# Autodesk Inventor assembly: protecaoAcrilico
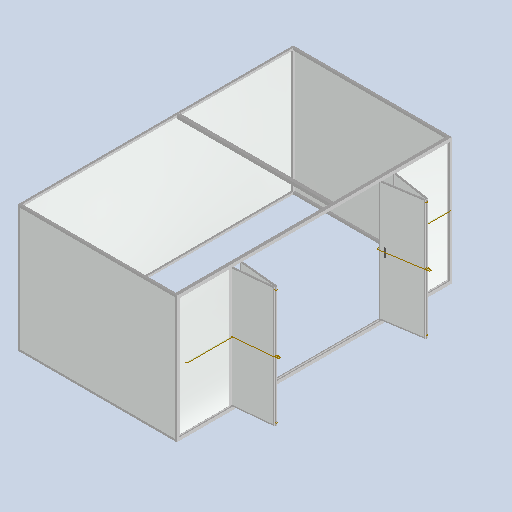
[picture p0: Inventor's stored thumbnail of the model, 512x512]
Saved by Autodesk Inventor 2023 (Build 270158000, 158)
## iProperties
Created: 2022-08-29
Part Number: protecaoAcrilico
Document SubType Name: Assembly
Designer: cvss2
Author: cvss2
## Documents named in this file (14)
- C:\Users\cvss2.CINSOFTEX\Documents\Residencia Softex 2021-2022\modelos 3D\Denso VS050\mesa2Denso\proteçao2Densos\protecaoAcrilico2Densos.iam
- C:\Users\cvss2.CINSOFTEX\Documents\Residencia Softex 2021-2022\modelos 3D\Denso VS050\mesa2Denso\proteçao2Densos\estrutura.ipt
- C:\Users\cvss2.CINSOFTEX\Documents\Residencia Softex 2021-2022\modelos 3D\Denso VS050\mesa2Denso\proteçao2Densos\acrilicoFixo.ipt
- C:\Users\cvss2.CINSOFTEX\Documents\Residencia Softex 2021-2022\modelos 3D\Denso VS050\mesa2Denso\proteçao2Densos\acrilicoFixo2.ipt
- C:\Users\cvss2.CINSOFTEX\Documents\Residencia Softex 2021-2022\modelos 3D\Denso VS050\mesa2Denso\proteçao2Densos\guiaPorta.ipt
- C:\Users\cvss2.CINSOFTEX\Documents\Residencia Softex 2021-2022\modelos 3D\Denso VS050\mesa2Denso\madeiraMesa.ipt
- C:\Users\cvss2.CINSOFTEX\Documents\Residencia Softex 2021-2022\modelos 3D\Denso VS050\mesa2Denso\proteçao2Densos\porta1.ipt
- C:\Users\cvss2.CINSOFTEX\Documents\Residencia Softex 2021-2022\modelos 3D\Denso VS050\mesa2Denso\proteçao2Densos\porta-2.ipt
- C:\Users\cvss2.CINSOFTEX\Documents\Residencia Softex 2021-2022\modelos 3D\Denso VS050\mesa2Denso\proteçao2Densos\corredor.ipt
- C:\Users\cvss2.CINSOFTEX\Documents\Residencia Softex 2021-2022\modelos 3D\Denso VS050\mesa2Denso\proteçao2Densos\acrilicoMovel1.ipt
- C:\Users\cvss2.CINSOFTEX\Documents\Residencia Softex 2021-2022\modelos 3D\Denso VS050\mesa2Denso\proteçao2Densos\acrilicoMovel2.ipt
- C:\Users\cvss2.CINSOFTEX\Documents\Residencia Softex 2021-2022\modelos 3D\Denso VS050\mesa2Denso\proteçao2Densos\apoioSuperior.ipt
- C:\Users\cvss2.CINSOFTEX\Documents\Residencia Softex 2021-2022\modelos 3D\Denso VS050\mesa2Denso\proteçao2Densos\porta-3.ipt
- C:\Users\cvss2.CINSOFTEX\Documents\Residencia Softex 2021-2022\modelos 3D\Denso VS050\mesa2Denso\proteçao2Densos\acrilicoFixo3.ipt
## Components (21 placed, 12 different names)
1. estrutura:1 — Flush:1, Mate:1, Mate:2, Flush:2, Mate:3, Mate:4, Flush:3, Mate:5, Mate:6, Flush:4, Mate:7, Flush:5, Flush:6, Mate:8, Flush:7, Flush:16, Mate:24, Mate:30
2. acrilicoFixo:1 — Flush:1, Mate:1, Mate:2
3. acrilicoFixo:2 — Flush:2, Mate:3, Mate:4
4. acrilicoFixo2:1 — Flush:3, Mate:5, Mate:6
5. guiaPorta:1 — Flush:4, Mate:7, Flush:5, Rotational:1, Slider:2, Slider:4
6. guiaPorta:2 — Flush:6, Mate:8, Flush:7, Slider:1, Rotational:4, Slider:3, Flush:17, Mate:23, Flush:20, Mate:29
7. porta1:1 — Rotational:1, Mate:9, Flush:8, Flush:9, Rotational:2, Flush:13, Mate:17, Mate:18
8. porta-2:1 — Mate:9, Flush:8, Flush:9, Slider:1, Rotational:2, Mate:10, Mate:11, Flush:15, Mate:21, Mate:22
9. corredor:1 — Mate:10, Mate:11, Slider:2
10. porta1:2 — Rotational:4, Flush:12, Mate:15, Mate:16
11. porta-2:2 — Flush:14, Mate:19, Mate:20
12. corredor:2 — Slider:3
13. acrilicoMovel1:1 — Flush:12, Mate:15, Mate:16
14. acrilicoMovel1:2 — Flush:13, Mate:17, Mate:18
15. acrilicoMovel2:1 — Flush:14, Mate:19, Mate:20
16. acrilicoMovel2:2 — Flush:15, Mate:21, Mate:22
17. apoioSuperior:1 — Flush:16, Slider:4
18. porta-3:1 — Flush:17, Mate:23, Mate:24, Flush:18, Mate:25, Mate:26
19. acrilicoFixo3:1 — Flush:18, Mate:25, Mate:26
20. porta-3:2 — Flush:20, Mate:29, Mate:30
21. acrilicoFixo3:2
## Relationships (58: Mate 30, Flush 20, RevoluteJoint 4, TranslationJoint 4)
- Flush:1: estrutura:1 ↔ acrilicoFixo:1
- Mate:1: estrutura:1 ↔ acrilicoFixo:1
- Mate:2: estrutura:1 ↔ acrilicoFixo:1
- Flush:2: estrutura:1 ↔ acrilicoFixo:2
- Mate:3: estrutura:1 ↔ acrilicoFixo:2
- Mate:4: estrutura:1 ↔ acrilicoFixo:2
- Flush:3: estrutura:1 ↔ acrilicoFixo2:1
- Mate:5: estrutura:1 ↔ acrilicoFixo2:1
- Mate:6: estrutura:1 ↔ acrilicoFixo2:1
- Flush:4: estrutura:1 ↔ guiaPorta:1
- Mate:7: estrutura:1 ↔ guiaPorta:1
- Flush:5: estrutura:1 ↔ guiaPorta:1
- Flush:6: estrutura:1 ↔ guiaPorta:2
- Mate:8: estrutura:1 ↔ guiaPorta:2
- Flush:7: estrutura:1 ↔ guiaPorta:2
- Rotational:1 [RevoluteJoint] (-1 mm): guiaPorta:1 ↔ porta1:1
- Mate:9: porta1:1 ↔ porta-2:1
- Flush:8: porta1:1 ↔ porta-2:1
- Flush:9: porta1:1 ↔ porta-2:1
- Slider:1 [TranslationJoint]: guiaPorta:2 ↔ porta-2:1
- Rotational:2 [RevoluteJoint]: porta1:1 ↔ porta-2:1
- Mate:10: porta-2:1 ↔ corredor:1
- Mate:11 (3 mm): porta-2:1 ↔ corredor:1
- Slider:2 [TranslationJoint] (13 mm): guiaPorta:1 ↔ corredor:1
- [Mate]: porta1:2 ↔ porta-2:2
- [Flush]: porta1:2 ↔ porta-2:2
- [Flush]: porta1:2 ↔ porta-2:2
- [RevoluteJoint]: porta1:2 ↔ porta-2:2
- [Mate]: porta-2:2 ↔ corredor:2
- [Mate] (3 mm): porta-2:2 ↔ corredor:2
- Rotational:4 [RevoluteJoint] (-1 mm): guiaPorta:2 ↔ porta1:2
- Slider:3 [TranslationJoint]: guiaPorta:2 ↔ corredor:2
- Flush:12 (2 mm): porta1:2 ↔ acrilicoMovel1:1
- Mate:15: porta1:2 ↔ acrilicoMovel1:1
- Mate:16: porta1:2 ↔ acrilicoMovel1:1
- Flush:13 (2 mm): porta1:1 ↔ acrilicoMovel1:2
- Mate:17: porta1:1 ↔ acrilicoMovel1:2
- Mate:18: porta1:1 ↔ acrilicoMovel1:2
- Flush:14 (2 mm): porta-2:2 ↔ acrilicoMovel2:1
- Mate:19: porta-2:2 ↔ acrilicoMovel2:1
- Mate:20: porta-2:2 ↔ acrilicoMovel2:1
- Flush:15 (2 mm): porta-2:1 ↔ acrilicoMovel2:2
- Mate:21: porta-2:1 ↔ acrilicoMovel2:2
- Mate:22: porta-2:1 ↔ acrilicoMovel2:2
- Flush:16: estrutura:1 ↔ apoioSuperior:1
- Slider:4 [TranslationJoint]: guiaPorta:1 ↔ apoioSuperior:1
- Flush:17 (10 mm): guiaPorta:2 ↔ porta-3:1
- Mate:23: guiaPorta:2 ↔ porta-3:1
- Mate:24 (8 mm): estrutura:1 ↔ porta-3:1
- Flush:18 (2 mm): porta-3:1 ↔ acrilicoFixo3:1
- Mate:25: porta-3:1 ↔ acrilicoFixo3:1
- Mate:26: porta-3:1 ↔ acrilicoFixo3:1
- [Flush] (2 mm): porta-3:2 ↔ acrilicoFixo3:2
- [Mate]: porta-3:2 ↔ acrilicoFixo3:2
- [Mate]: porta-3:2 ↔ acrilicoFixo3:2
- Flush:20 (10 mm): guiaPorta:2 ↔ porta-3:2
- Mate:29 (1 mm): guiaPorta:2 ↔ porta-3:2
- Mate:30 (8 mm): estrutura:1 ↔ porta-3:2
## Named parameters: largura = 2600 mm, comprimento = 1500 mm, d36_d23 = 0 mm, d37_d24 = 0 mm, d38_d25 = 0 mm, d39_d28 = 0 mm, d40_d29 = 168.902844 deg, d41_d30 = 0 mm, d42_d31 = 3 mm, d75_d72 = 2 mm, d76_d73 = 0 mm, d77_d74 = 0 mm
